# Autodesk Inventor assembly: Intake Bumper1
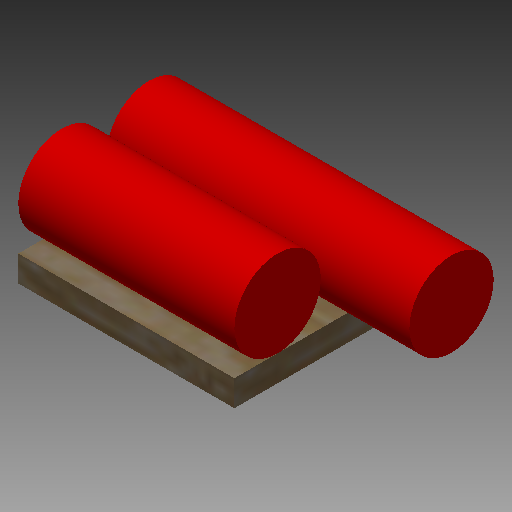
[picture p0: Inventor's stored thumbnail of the model, 512x512]
Saved by Autodesk Inventor 2018 (Build 220112000, 112)
## iProperties
Created: 2018-01-17
Part Number: Intake Bumper1
Document SubType Name: Assembly
Designer: Apple
Author: Apple
## Documents named in this file (4)
- C:\Users\Apple\Documents\Inventor\2018 PowerUp\Bumper\Intake Bumper1.iam
- C:\Users\Apple\Documents\Inventor\2018 PowerUp\Bumper\3_4 Intake Board.ipt
- C:\Users\Apple\Documents\Inventor\2018 PowerUp\Bumper\Intake Noodle Long.ipt
- C:\Users\Apple\Documents\Inventor\2018 PowerUp\Bumper\Short Noodle.ipt
## Components (3 placed, 3 different names)
1. 3_4 Intake Board:1 — Flush:1, Flush:2
2. Intake Noodle Long:1 — Flush:1
3. Short Noodle:1 — Flush:2
## Relationships (2: Flush 2)
- Flush:1: 3_4 Intake Board:1 ↔ Intake Noodle Long:1
- Flush:2: 3_4 Intake Board:1 ↔ Short Noodle:1
